# Autodesk Inventor assembly: Assembled
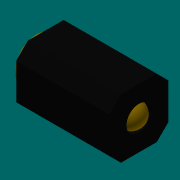
[picture p0: Inventor's stored thumbnail of the model, 180x180]
Saved by Autodesk Inventor 2016 (Build 200138000, 138)
## iProperties
Created: 2016-05-20
Part Number: Assembled
Document SubType Name: Assembly
Designer: Jonathan
Author: Jonathan
## Documents named in this file (3)
- C:\Users\sawaiz\oneDrive\projects\splitFlapDisplay\electronics\cad\component\Preci-Dip 811\Assembled.iam
- C:\Users\sawaiz\oneDrive\projects\splitFlapDisplay\electronics\cad\component\Preci-Dip 811\body.ipt
- C:\Users\sawaiz\oneDrive\projects\splitFlapDisplay\electronics\cad\component\Preci-Dip 811\pin.ipt
## Components (2 placed, 2 different names)
1. pin:1 — Mate:1, Mate:2, Flush:1
2. body:1 — Mate:1, Mate:2, Flush:1
## Relationships (3: Mate 2, Flush 1)
- Mate:1: pin:1 ↔ body:1
- Mate:2: pin:1 ↔ body:1
- Flush:1 (2 mm): pin:1 ↔ body:1
